# Autodesk Inventor assembly: 부피 구하기
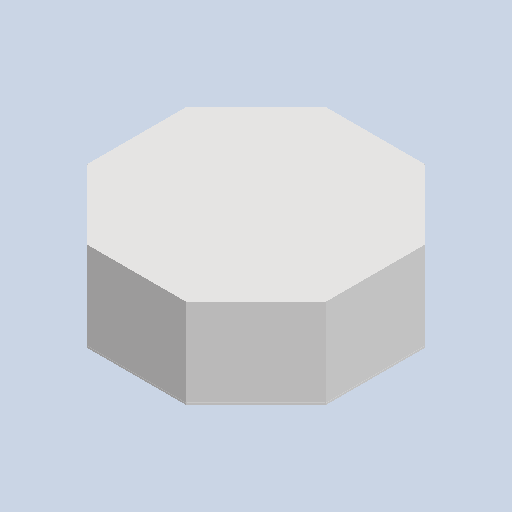
[picture p0: Inventor's stored thumbnail of the model, 512x512]
Saved by Autodesk Inventor 2024 (Build 280153000, 153)
## iProperties
Created: 2023-06-26
Part Number: 부피 구하기
Document SubType Name: Assembly
Designer: jsw
Author: jsw
## Documents named in this file (3)
- C:\승원\co-op\OV-PAM\OV-PAM_modeling\부피 구하기.iam
- C:\승원\co-op\OV-PAM\OV-PAM_modeling\OV-PAM_5_patterns_1f 부피 구하기 60도 - 복사본.ipt
- C:\승원\co-op\OV-PAM\OV-PAM_modeling\OV-PAM_5_patterns_1f 부피 구하기 60도.ipt
## Components (2 placed, 2 different names)
1. OV-PAM_5_patterns_1f 부피 구하기 60도 - 복사본:1 — 플러쉬:1, 메이트:1, 메이트:2
2. OV-PAM_5_patterns_1f 부피 구하기 60도:1 — 플러쉬:1, 메이트:1, 메이트:2
## Relationships (3: Mate 2, Flush 1)
- 플러쉬:1 [Flush]: OV-PAM_5_patterns_1f 부피 구하기 60도 - 복사본:1 ↔ OV-PAM_5_patterns_1f 부피 구하기 60도:1
- 메이트:1 [Mate]: OV-PAM_5_patterns_1f 부피 구하기 60도 - 복사본:1 ↔ OV-PAM_5_patterns_1f 부피 구하기 60도:1
- 메이트:2 [Mate]: OV-PAM_5_patterns_1f 부피 구하기 60도 - 복사본:1 ↔ OV-PAM_5_patterns_1f 부피 구하기 60도:1
